# Autodesk Inventor assembly: DC_motor
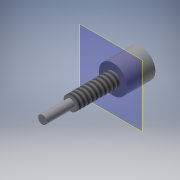
[picture p0: Inventor's stored thumbnail of the model, 180x180]
Saved by Autodesk Inventor 2019 (Build 230136000, 136)
## iProperties
Created: 2020-02-29
Part Number: DC_motor
Document SubType Name: Assembly
Designer: Prajwal
Author: Prajwal
## Documents named in this file (3)
- C:\Users\Prajwal\Documents\DC_motor.iam
- C:\Users\Prajwal\Documents\DC1.ipt
- C:\Users\Prajwal\Documents\DC2.ipt
## Components (2 placed, 2 different names)
1. DC1:1 — Flush:1
2. DC2:2 — Flush:1
## Relationships (1: Flush 1)
- Flush:1: DC1:1 ↔ DC2:2
